# Autodesk Inventor assembly: Cart
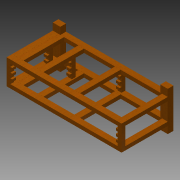
[picture p0: Inventor's stored thumbnail of the model, 180x180]
Saved by Autodesk Inventor 2014 SP1 (Build 180222100, 222)
## iProperties
Created: 2014-02-22
Part Number: Cart
Document SubType Name: Assembly
Designer: tuleu
Author: tuleu
## Documents named in this file (6)
- C:\Users\tuleu\Documents\giant-snes-gamepad\cad\Cart\Cart.iam
- C:\Users\tuleu\Documents\giant-snes-gamepad\cad\Cart\Separator.ipt
- C:\Users\tuleu\Documents\giant-snes-gamepad\cad\Cart\Transverse_High.ipt
- C:\Users\tuleu\Documents\giant-snes-gamepad\cad\Cart\Tower_Out.ipt
- C:\Users\tuleu\Documents\giant-snes-gamepad\cad\Cart\Bottom_Wheel_Supp.ipt
- C:\Users\tuleu\Documents\giant-snes-gamepad\cad\Cart\Transverse_Bottom.ipt
## Components (21 placed, 5 different names)
1. Separator:1 — Flush:1, Flush:2, Mate:1, Flush:3, Flush:4, Flush:5, Flush:6, Flush:7, Mate:2, Mate:3
2. Separator:2 — Flush:1, Flush:2, Mate:1, Flush:28
3. Separator:3 — Flush:3, Flush:4, Flush:5, Flush:25, Mate:11, Flush:31
4. Separator:4 — Flush:6, Flush:8, Mate:4
5. Separator:5 — Flush:7, Mate:2, Mate:3, Flush:8, Mate:4, Flush:9, Flush:10, Mate:5, Flush:11, Flush:12, Mate:6
6. Transverse_High:1 — Flush:9, Flush:10, Mate:5, Flush:13, Mate:9, Flush:19, Flush:20, Flush:27, Mate:15, Flush:29, Flush:30
7. Transverse_High:2 — Flush:11, Flush:12, Mate:6, Flush:15, Mate:7, Flush:16, Flush:17, Mate:8, Flush:18, Flush:32, Flush:34, Flush:36
8. Tower_Out:1 — Flush:13, Flush:14, Mate:14
9. Bottom_Wheel_Supp:1 — Flush:14, Flush:21, Flush:22, Mate:10, Flush:23
10. Tower_Out:2 — Flush:15, Mate:7, Flush:16, Mate:10, Flush:23, Mate:20
11. Tower_Out:3 — Flush:17, Mate:8, Flush:18
12. Tower_Out:4 — Mate:9, Flush:19, Flush:20, Flush:24
13. Bottom_Wheel_Supp:2 — Flush:21, Flush:22, Flush:24, Mate:12, Flush:26
14. Transverse_Bottom:1 — Flush:25, Mate:13, Mate:16
15. Transverse_Bottom:2 — Mate:11, Mate:12, Flush:26, Mate:17, Mate:18, Mate:19
16. Tower_Out:5 — Flush:32, Mate:17, Flush:33
17. Tower_Out:6 — Mate:18, Flush:34, Flush:35
18. Tower_Out:7 — Flush:36, Mate:19, Mate:20
19. Tower_Out:8 — Flush:27, Mate:13, Mate:14
20. Tower_Out:9 — Mate:15, Flush:28, Flush:29, Flush:35
21. Tower_Out:10 — Flush:30, Mate:16, Flush:31, Flush:33
## Relationships (56: Flush 36, Mate 20)
- Flush:1: Separator:1 ↔ Separator:2
- Flush:2: Separator:1 ↔ Separator:2
- Mate:1 (200 mm): Separator:1 ↔ Separator:2
- Flush:3: Separator:1 ↔ Separator:3
- Flush:4 (-140 mm): Separator:1 ↔ Separator:3
- Flush:5 (630 mm): Separator:1 ↔ Separator:3
- Flush:6: Separator:1 ↔ Separator:4
- Flush:7: Separator:1 ↔ Separator:5
- Mate:2 (333 mm): Separator:1 ↔ Separator:5
- Mate:3 (3 mm): Separator:1 ↔ Separator:5
- Flush:8: Separator:4 ↔ Separator:5
- Mate:4 (1146 mm): Separator:4 ↔ Separator:5
- Flush:9: Separator:5 ↔ Transverse_High:1
- Flush:10: Separator:5 ↔ Transverse_High:1
- Mate:5: Separator:5 ↔ Transverse_High:1
- Flush:11: Separator:5 ↔ Transverse_High:2
- Flush:12: Separator:5 ↔ Transverse_High:2
- Mate:6: Separator:5 ↔ Transverse_High:2
- Flush:13: Transverse_High:1 ↔ Tower_Out:1
- Flush:14: Tower_Out:1 ↔ Bottom_Wheel_Supp:1
- Flush:15: Transverse_High:2 ↔ Tower_Out:2
- Mate:7: Transverse_High:2 ↔ Tower_Out:2
- Flush:16: Transverse_High:2 ↔ Tower_Out:2
- Flush:17: Transverse_High:2 ↔ Tower_Out:3
- Mate:8: Transverse_High:2 ↔ Tower_Out:3
- Flush:18: Transverse_High:2 ↔ Tower_Out:3
- Mate:9: Transverse_High:1 ↔ Tower_Out:4
- Flush:19: Transverse_High:1 ↔ Tower_Out:4
- Flush:20: Transverse_High:1 ↔ Tower_Out:4
- Flush:21: Bottom_Wheel_Supp:1 ↔ Bottom_Wheel_Supp:2
- Flush:22: Bottom_Wheel_Supp:1 ↔ Bottom_Wheel_Supp:2
- Mate:10: Bottom_Wheel_Supp:1 ↔ Tower_Out:2
- Flush:23: Bottom_Wheel_Supp:1 ↔ Tower_Out:2
- Flush:24: Tower_Out:4 ↔ Bottom_Wheel_Supp:2
- Flush:25: Separator:3 ↔ Transverse_Bottom:1
- Mate:11: Separator:3 ↔ Transverse_Bottom:2
- Mate:12: Bottom_Wheel_Supp:2 ↔ Transverse_Bottom:2
- Flush:26: Bottom_Wheel_Supp:2 ↔ Transverse_Bottom:2
- Flush:27: Transverse_High:1 ↔ Tower_Out:8
- Mate:13: Transverse_Bottom:1 ↔ Tower_Out:8
- Mate:14: Tower_Out:1 ↔ Tower_Out:8
- Mate:15: Transverse_High:1 ↔ Tower_Out:9
- Flush:28 (-10 mm): Separator:2 ↔ Tower_Out:9
- Flush:29: Transverse_High:1 ↔ Tower_Out:9
- Flush:30: Transverse_High:1 ↔ Tower_Out:10
- Mate:16: Transverse_Bottom:1 ↔ Tower_Out:10
- Flush:31 (-10 mm): Separator:3 ↔ Tower_Out:10
- Flush:32: Transverse_High:2 ↔ Tower_Out:5
- Mate:17: Transverse_Bottom:2 ↔ Tower_Out:5
- Flush:33: Tower_Out:5 ↔ Tower_Out:10
- Mate:18: Transverse_Bottom:2 ↔ Tower_Out:6
- Flush:34: Transverse_High:2 ↔ Tower_Out:6
- Flush:35: Tower_Out:6 ↔ Tower_Out:9
- Flush:36: Transverse_High:2 ↔ Tower_Out:7
- Mate:19: Transverse_Bottom:2 ↔ Tower_Out:7
- Mate:20: Tower_Out:2 ↔ Tower_Out:7
